# Autodesk Inventor assembly: Tensioner
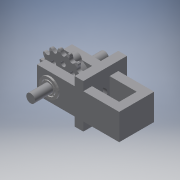
[picture p0: Inventor's stored thumbnail of the model, 180x180]
Saved by Autodesk Inventor 2017 (Build 210142000, 142)
## iProperties
Created: 2017-07-29
Part Number: Tensioner
Document SubType Name: Assembly
Designer: User
Author: User
## Documents named in this file (7)
- C:\Robotics\CAD\2016-17_CAD\DriveTrain\Tensioner.iam
- C:\Robotics\CAD\2016-17_CAD\DriveTrain\TensionerAxleHolder.ipt
- C:\Robotics\CAD\2016-17_CAD\DriveTrain\TensionerPlate.ipt
- C:\Robotics\CAD\COTSParts\Bearings - AndyMark\Bearing 250 ID 500 OD flanged_MIR.ipt
- C:\Robotics\CAD\2016-17_CAD\Custom COTS\Axle2.11.ipt
- C:\Robotics\CAD\COTSParts\Actobotics\615 parts\615102.ipt
- C:\Robotics\CAD\COTSParts\Actobotics\545 parts\545556.ipt
## Components (7 placed, 6 different names)
1. TensionerAxleHolder:1 — Mate:1, Flush:1, Insert:1, Insert:2, Insert:3, Insert:4, Flush:2
2. TensionerPlate:1 — Mate:1, Flush:1, Flush:2
3. Bearing 250 ID 500 OD flanged_MIR:1 — Insert:1
4. Bearing 250 ID 500 OD flanged_MIR:2 — Insert:2
5. Axle2.11:1 — Insert:3
6. 615102:1 — Insert:4, Insert:5
7. 545556:1 — Insert:5
## Relationships (8: Insert 5, Flush 2, Mate 1)
- Mate:1: TensionerAxleHolder:1 ↔ TensionerPlate:1
- Flush:1 (6.35 mm): TensionerAxleHolder:1 ↔ TensionerPlate:1
- Insert:1: TensionerAxleHolder:1 ↔ Bearing 250 ID 500 OD flanged_MIR:1
- Insert:2: TensionerAxleHolder:1 ↔ Bearing 250 ID 500 OD flanged_MIR:2
- Insert:3 (-14.097 mm): TensionerAxleHolder:1 ↔ Axle2.11:1
- Insert:4 (3.175 mm): TensionerAxleHolder:1 ↔ 615102:1
- Insert:5: 615102:1 ↔ 545556:1
- Flush:2 (-26.035 mm): TensionerAxleHolder:1 ↔ TensionerPlate:1
